# Autodesk Inventor assembly: bumper
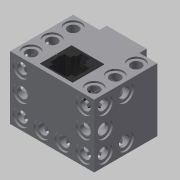
[picture p0: Inventor's stored thumbnail of the model, 180x180]
Saved by Autodesk Inventor 2019.3 (Build 233278000, 278)
## iProperties
Created: 2019-02-12
Part Number: bumper
Document SubType Name: Assembly
Designer: Varga Daniel
Author: Varga Daniel
## Documents named in this file (8)
- C:\!_Dani\!_cloud\OneDrive\!_munka\Revolution\RevvyDemoKit\Structural parts\Demo parts\Bumper\Inventor imported\bumper.iam
- C:\!_Dani\!_cloud\OneDrive\!_munka\Revolution\RevvyDemoKit\Structural parts\Demo parts\Bumper\Inventor imported\ressort.ipt
- C:\!_Dani\!_cloud\OneDrive\!_munka\Revolution\RevvyDemoKit\Structural parts\Demo parts\Bumper\Inventor imported\omron b3w-4000 switch.ipt
- C:\!_Dani\!_cloud\OneDrive\!_munka\Revolution\RevvyDemoKit\Structural parts\Connetor Pins\CP1+x1+\CP1x1.ipt
- C:\!_Dani\!_cloud\OneDrive\!_munka\Revolution\RevvyDemoKit\Structural parts\Demo parts\Bumper\Inventor imported\RJ45 - MTJ-881X1.ipt
- C:\!_Dani\!_cloud\OneDrive\!_munka\Revolution\RevvyDemoKit\Structural parts\Demo parts\Bumper\Inventor imported\BUcA_1.ipt
- C:\!_Dani\!_cloud\OneDrive\!_munka\Revolution\RevvyDemoKit\Structural parts\Demo parts\Bumper\Inventor imported\BUcA_3.ipt
- C:\!_Dani\!_cloud\OneDrive\!_munka\Revolution\RevvyDemoKit\Structural parts\Demo parts\Bumper\Inventor imported\BUcA_2.ipt
## Components (8 placed, 7 different names)
1. ressort:1 — Mate:8, Mate:9, Mate:10
2. CP1x1:1 — Insert:1
3. BUcA_1:1 — Mate:6, Flush:11, Flush:12, Flush:13, Flush:14, Mate:11, Insert:2, Mate:17, Mate:18, Flush:16
4. BUcA_3:1 — Insert:1, Mate:6, Mate:8, Mate:9, Mate:10, Flush:11, Mate:11, Mate:12, Flush:15
5. RJ45 - MTJ-881X1:1 — Flush:12, Flush:13, Flush:14, Tangent:1
6. CP1x1:2 — Insert:2
7. omron b3w-4000 switch:1 — Mate:12, Flush:15, Tangent:1
8. BUcA_2:1 — Mate:17, Mate:18, Flush:16
## Relationships (17: Mate 8, Flush 6, Insert 2, Tangent 1)
- Insert:1: CP1x1:1 ↔ BUcA_3:1
- Mate:6: BUcA_1:1 ↔ BUcA_3:1
- Mate:8: ressort:1 ↔ BUcA_3:1
- Mate:9: ressort:1 ↔ BUcA_3:1
- Mate:10: ressort:1 ↔ BUcA_3:1
- Flush:11 (-6 mm): BUcA_1:1 ↔ BUcA_3:1
- Flush:12 (2 mm): BUcA_1:1 ↔ RJ45 - MTJ-881X1:1
- Flush:13: BUcA_1:1 ↔ RJ45 - MTJ-881X1:1
- Flush:14: BUcA_1:1 ↔ RJ45 - MTJ-881X1:1
- Mate:11: BUcA_1:1 ↔ BUcA_3:1
- Insert:2: BUcA_1:1 ↔ CP1x1:2
- Mate:12: BUcA_3:1 ↔ omron b3w-4000 switch:1
- Flush:15: BUcA_3:1 ↔ omron b3w-4000 switch:1
- Tangent:1 (2 mm): RJ45 - MTJ-881X1:1 ↔ omron b3w-4000 switch:1
- Mate:17 (-30 mm): BUcA_1:1 ↔ BUcA_2:1
- Mate:18: BUcA_1:1 ↔ BUcA_2:1
- Flush:16: BUcA_1:1 ↔ BUcA_2:1
